# Autodesk Inventor assembly: Assembly1
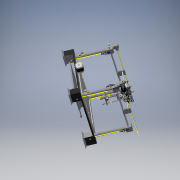
[picture p0: Inventor's stored thumbnail of the model, 180x180]
Saved by Autodesk Inventor 2017 (Build 210142000, 142)
## iProperties
Created: 2018-11-09
Part Number: Assembly1
Document SubType Name: Assembly
Designer: Antoine Blaud
Author: Antoine Blaud
## Documents named in this file (23)
- D:\Document\C\Arduino\project\pièces\Assembly1.iam
- D:\Document\C\Arduino\project\pièces\planche.ipt
- D:\Document\C\Arduino\project\pièces\cylindre1.ipt
- D:\Document\C\Arduino\project\pièces\barre latérales.ipt
- D:\Document\C\Arduino\project\pièces\coulissant coté.ipt
- D:\Document\C\Arduino\project\pièces\cube fixation2.ipt
- D:\Document\C\Arduino\project\pièces\barre horizontaleipt.ipt
- D:\Document\C\Arduino\project\pièces\Download\M1173041- NEMA 17.ipt
- D:\Document\C\Arduino\project\pièces\petit\barre filté.ipt
- D:\Document\C\Arduino\project\pièces\petit\planche.ipt
- D:\Document\C\Arduino\project\pièces\petit\pied.ipt
- D:\Document\C\Arduino\project\pièces\petit\rails.ipt
- D:\Document\C\Arduino\project\pièces\petit\rond tournant 1.ipt
- D:\Document\C\Arduino\project\pièces\petit\rond tournant 2.ipt
- D:\Document\C\Arduino\project\pièces\petit\repose rond tournant 1.ipt
- D:\Document\C\Arduino\project\pièces\plateform.ipt
- D:\Document\C\Arduino\project\pièces\petit\cylindre plateform.ipt
- D:\Document\C\Arduino\project\pièces\petit\plateform du bas.ipt
- D:\Document\C\Arduino\project\pièces\petit\bout stylo.ipt
- D:\Document\C\Arduino\project\pièces\Part10.ipt
- D:\Document\C\Arduino\project\pièces\petit\roue denté 3.ipt
- D:\Document\C\Arduino\project\pièces\petit\stylo assemblé.iam
- D:\Document\C\Arduino\project\pièces\petit\barre filté 2.ipt
## Components (49 placed, 21 different names)
1. planche:1 — Insert:1, Insert:2, Insert:4, Insert:6, Angle:1, Angle:2, Angle:3, Angle:4, Mate:24, Mate:25, Mate:26, Mate:27, Mate:28, Mate:29, Mate:30, Mate:31, Mate:32, Mate:33, Mate:34, Mate:35, Flush:1, Mate:42, Angle:6, Angle:7, Mate:52, Mate:53, Mate:54, Mate:55, Mate:56, Angle:8, Mate:60, Flush:7, Flush:8, Flush:12, Flush:13
2. cylindre1:1 — Insert:1, Insert:9, Flush:2, Flush:3, Mate:44, Angle:6, Mate:45, Mate:46, Mate:47, Mate:48
3. cylindre1:2 — Insert:2, Insert:10
4. cylindre1:4 — Insert:4, Insert:8, Angle:7, Mate:49, Flush:4, Mate:50, Mate:51
5. cylindre1:5 — Insert:6, Insert:7
6. cube fixation2:1 — Insert:8, Angle:1, Mate:1, Mate:2, Symmetry:1, Mate:20, Flush:5, Angle:10
7. cube fixation2:2 — Insert:10, Angle:4, Mate:5, Mate:6, Mate:7, Mate:8
8. cube fixation2:3 — Insert:9, Angle:2, Symmetry:1, Mate:21, Flush:6, Angle:9, Mate:62, Mate:63
9. cube fixation2:4 — Insert:7, Angle:3, Mate:3, Mate:4
10. barre latérales:1 — Mate:7, Mate:8, Mate:11
11. barre latérales:2 — Mate:5, Mate:6, Mate:12
12. barre latérales:3 — Mate:3, Mate:4, Mate:10
13. barre latérales:4 — Mate:1, Mate:2, Mate:9
14. coulissant coté:1 — Mate:9, Mate:10, Symmetry:2, Mate:14, Mate:15, Mate:16, Mate:17, Mate:19, Rotation/Translation:2, Mate:80
15. coulissant coté:2 — Mate:11, Mate:12, Symmetry:2, Mate:13, Mate:18, Rotation/Translation:1
16. barre horizontaleipt:1 — Mate:13, Mate:14, Mate:15, Mate:66
17. barre horizontaleipt:2 — Mate:16, Mate:17, Mate:65
18. M1173041- NEMA 17:1 — Mate:60, Flush:7, Flush:8
19. barre filté:1 — Mate:19, Mate:20, Rotation/Translation:2, Mate:58
20. barre filté:2 — Mate:18, Rotation/Translation:1, Mate:21, Mate:59
21. pied:1 — Mate:27, Mate:28, Mate:29
22. pied:2 — Mate:26, Mate:30, Mate:31
23. pied:3 — Mate:25, Mate:34, Mate:35
24. pied:4 — Mate:24, Mate:32, Mate:33
25. rails:1 — Flush:1, Mate:52, Mate:53, Mate:56
26. rails:2 — Mate:42, Mate:54, Mate:55, Mate:57
27. rond tournant 1:1 — Mate:44, Mate:45, Mate:46
28. rond tournant 1:2 — Mate:49, Flush:4, Rotation:1
29. rond tournant 1:3 — Mate:50, Mate:51, Rotation:1
30. rond tournant 1:4 — Mate:47, Mate:48
31. planche:2 — Mate:57, Angle:8
32. rond tournant 2:1 — Mate:58, Flush:5, Mate:64
33. rond tournant 2:2 — Mate:59, Flush:6, Mate:61
34. repose rond tournant 1:1 — Mate:61, Angle:9, Mate:62, Mate:63
35. repose rond tournant 1:2 — Mate:64, Angle:10
36. plateform:1 — Mate:65, Mate:66, Mate:67, Mate:68, Mate:69, Mate:70, Mate:71, Mate:72, Mate:73, Mate:74, Mate:78, Flush:9, Mate:81, Angle:11, Mate:82, Flush:10, Mate:83, Flush:11, Mate:84
37. cylindre plateform:1 — Mate:69, Mate:74
38. cylindre plateform:2 — Mate:70, Mate:73, Mate:76
39. cylindre plateform:3 — Mate:71, Mate:72, Mate:75
40. cylindre plateform:4 — Mate:67, Mate:68, Mate:77, Mate:79
41. plateform du bas:1 — Mate:75, Mate:76, Mate:77, Mate:78, Mate:87, Mate:88
42. M1173041- NEMA 17:2 — Mate:79, Mate:80, Flush:9, Mate:85
43. bout stylo:1
44. Part10:1 — Mate:87, Mate:88
45. roue denté 3:1 — Mate:81, Angle:11, Flush:11
46. stylo assemblé:1 [sub-assembly] — Mate:82, Flush:10, Mate:83
47. barre filté 2:1 — Mate:84, Flush:12, Mate:86
48. roue denté 3:2 — Mate:85
49. roue denté 3:3 — Mate:86, Flush:13
## Relationships (115: Mate 79, Flush 13, Angle 10, Insert 8, Symmetry 2, RelateRotateTranslate 2, RelateRotation 1)
- Insert:1: planche:1 ↔ cylindre1:1
- Insert:2: planche:1 ↔ cylindre1:2
- Insert:4: planche:1 ↔ cylindre1:4
- Insert:6: planche:1 ↔ cylindre1:5
- Insert:7: cylindre1:5 ↔ cube fixation2:4
- Insert:8: cylindre1:4 ↔ cube fixation2:1
- Insert:9: cylindre1:1 ↔ cube fixation2:3
- Insert:10: cylindre1:2 ↔ cube fixation2:2
- Angle:1 (0 deg): planche:1 ↔ cube fixation2:1
- Angle:2 (0 deg): planche:1 ↔ cube fixation2:3
- Angle:3 (0 deg): planche:1 ↔ cube fixation2:4
- Angle:4 (0 deg): planche:1 ↔ cube fixation2:2
- Mate:1: cube fixation2:1 ↔ barre latérales:4
- Mate:2 (6.35 mm): cube fixation2:1 ↔ barre latérales:4
- Mate:3: cube fixation2:4 ↔ barre latérales:3
- Mate:4 (6.35 mm): cube fixation2:4 ↔ barre latérales:3
- Mate:5: cube fixation2:2 ↔ barre latérales:2
- Mate:6 (6.35 mm): cube fixation2:2 ↔ barre latérales:2
- Mate:7: cube fixation2:2 ↔ barre latérales:1
- Mate:8 (6.35 mm): cube fixation2:2 ↔ barre latérales:1
- Mate:9: barre latérales:4 ↔ coulissant coté:1
- Mate:10: barre latérales:3 ↔ coulissant coté:1
- Mate:11: barre latérales:1 ↔ coulissant coté:2
- Mate:12: barre latérales:2 ↔ coulissant coté:2
- Symmetry:1: cube fixation2:1 ↔ cube fixation2:3
- Symmetry:2: coulissant coté:1 ↔ coulissant coté:2
- Mate:13: coulissant coté:2 ↔ barre horizontaleipt:1
- Mate:14: coulissant coté:1 ↔ barre horizontaleipt:1
- Mate:15: coulissant coté:1 ↔ barre horizontaleipt:1
- Mate:16: coulissant coté:1 ↔ barre horizontaleipt:2
- Mate:17: coulissant coté:1 ↔ barre horizontaleipt:2
- Mate:18: coulissant coté:2 ↔ barre filté:2
- Rotation/Translation:1 [RelateRotateTranslate] (1 mm): coulissant coté:2 ↔ barre filté:2
- Mate:19: coulissant coté:1 ↔ barre filté:1
- Mate:20: cube fixation2:1 ↔ barre filté:1
- Rotation/Translation:2 [RelateRotateTranslate] (11.9634 mm): coulissant coté:1 ↔ barre filté:1
- Mate:21: cube fixation2:3 ↔ barre filté:2
- Mate:24: planche:1 ↔ pied:4
- Mate:25: planche:1 ↔ pied:3
- Mate:26: planche:1 ↔ pied:2
- Mate:27: planche:1 ↔ pied:1
- Mate:28: planche:1 ↔ pied:1
- Mate:29: planche:1 ↔ pied:1
- Mate:30: planche:1 ↔ pied:2
- Mate:31 (0.0762 mm): planche:1 ↔ pied:2
- Mate:32: planche:1 ↔ pied:4
- Mate:33: planche:1 ↔ pied:4
- Mate:34: planche:1 ↔ pied:3
- Mate:35: planche:1 ↔ pied:3
- Flush:1: planche:1 ↔ rails:1
- Mate:42: planche:1 ↔ rails:2
- Flush:2: cylindre1:1
- Flush:3: cylindre1:1
- Mate:44: cylindre1:1 ↔ rond tournant 1:1
- Angle:6 (270 deg): planche:1 ↔ cylindre1:1
- Angle:7 (90 deg): planche:1 ↔ cylindre1:4
- Mate:45: cylindre1:1 ↔ rond tournant 1:1
- Mate:46 (18 mm): cylindre1:1 ↔ rond tournant 1:1
- Mate:47: cylindre1:1 ↔ rond tournant 1:4
- Mate:48 (18 mm): cylindre1:1 ↔ rond tournant 1:4
- Mate:49: cylindre1:4 ↔ rond tournant 1:2
- Flush:4 (18 mm): cylindre1:4 ↔ rond tournant 1:2
- Mate:50: cylindre1:4 ↔ rond tournant 1:3
- Mate:51 (-18 mm): cylindre1:4 ↔ rond tournant 1:3
- Mate:52 (-5 mm): planche:1 ↔ rails:1
- Mate:53: planche:1 ↔ rails:1
- Mate:54: planche:1 ↔ rails:2
- Mate:55 (30 mm): planche:1 ↔ rails:2
- Mate:56 (30 mm): planche:1 ↔ rails:1
- Mate:57: rails:2 ↔ planche:2
- Angle:8 (180 deg): planche:1 ↔ planche:2
- Rotation:1 [RelateRotation] (1 ul): rond tournant 1:2 ↔ rond tournant 1:3
- Mate:58: barre filté:1 ↔ rond tournant 2:1
- Flush:5 (-12 mm): cube fixation2:1 ↔ rond tournant 2:1
- Mate:59: barre filté:2 ↔ rond tournant 2:2
- Flush:6 (-12 mm): cube fixation2:3 ↔ rond tournant 2:2
- Mate:60: planche:1 ↔ M1173041- NEMA 17:1
- Flush:7 (-40 mm): planche:1 ↔ M1173041- NEMA 17:1
- Flush:8 (-150 mm): planche:1 ↔ M1173041- NEMA 17:1
- Mate:61: rond tournant 2:2 ↔ repose rond tournant 1:1
- Angle:9 (180 deg): cube fixation2:3 ↔ repose rond tournant 1:1
- Mate:62: cube fixation2:3 ↔ repose rond tournant 1:1
- Mate:63: cube fixation2:3 ↔ repose rond tournant 1:1
- Mate:64: rond tournant 2:1 ↔ repose rond tournant 1:2
- Angle:10 (180 deg): cube fixation2:1 ↔ repose rond tournant 1:2
- Mate:65: barre horizontaleipt:2 ↔ plateform:1
- Mate:66: barre horizontaleipt:1 ↔ plateform:1
- Mate:67: plateform:1 ↔ cylindre plateform:4
- Mate:68: plateform:1 ↔ cylindre plateform:4
- Mate:69: plateform:1 ↔ cylindre plateform:1
- Mate:70: plateform:1 ↔ cylindre plateform:2
- Mate:71: plateform:1 ↔ cylindre plateform:3
- Mate:72: plateform:1 ↔ cylindre plateform:3
- Mate:73: plateform:1 ↔ cylindre plateform:2
- Mate:74: plateform:1 ↔ cylindre plateform:1
- Mate:75: cylindre plateform:3 ↔ plateform du bas:1
- Mate:76: cylindre plateform:2 ↔ plateform du bas:1
- Mate:77: cylindre plateform:4 ↔ plateform du bas:1
- Mate:78 (114.3 mm): plateform:1 ↔ plateform du bas:1
- Mate:79 (-38.1 mm): cylindre plateform:4 ↔ M1173041- NEMA 17:2
- Mate:80 (120.396 mm): coulissant coté:1 ↔ M1173041- NEMA 17:2
- Flush:9 (55 mm): plateform:1 ↔ M1173041- NEMA 17:2
- Mate:81 (25.4 mm): plateform:1 ↔ roue denté 3:1
- Angle:11 (0 deg): plateform:1 ↔ roue denté 3:1
- Mate:82 (25.4 mm): plateform:1 ↔ stylo assemblé:1
- Flush:10 (12.25 mm): plateform:1 ↔ stylo assemblé:1
- Mate:83 (13 mm): plateform:1 ↔ stylo assemblé:1
- Flush:11 (-5 mm): plateform:1 ↔ roue denté 3:1
- Mate:84: plateform:1 ↔ barre filté 2:1
- Flush:12 (-279.4 mm): planche:1 ↔ barre filté 2:1
- Mate:85: M1173041- NEMA 17:2 ↔ roue denté 3:2
- Mate:86: barre filté 2:1 ↔ roue denté 3:3
- Flush:13 (-264.16 mm): planche:1 ↔ roue denté 3:3
- Mate:87: plateform du bas:1 ↔ Part10:1
- Mate:88 (-45.72 mm): plateform du bas:1 ↔ Part10:1
